# Autodesk Inventor assembly: Assembly
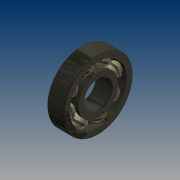
[picture p0: Inventor's stored thumbnail of the model, 180x180]
Saved by Autodesk Inventor 2014 (Build 180170000, 170)
## iProperties
Created: 2021-03-19
Part Number: Assembly
Document SubType Name: Assembly
Designer: Think Station
Author: Think Station
## Documents named in this file (5)
- E:\Entraco_Diptanshu\3D\##TEST##\Ball Bearing\Assembly.iam
- E:\Entraco_Diptanshu\3D\##TEST##\Ball Bearing\Outer Ring.ipt
- E:\Entraco_Diptanshu\3D\##TEST##\Ball Bearing\Inner Ring.ipt
- E:\Entraco_Diptanshu\3D\##TEST##\Ball Bearing\Ball.ipt
- E:\Entraco_Diptanshu\3D\##TEST##\Ball Bearing\Cage.ipt
## Components (12 placed, 4 different names)
1. Outer Ring:1 — Mate:1, Mate:2, Flush:1
2. Inner Ring:1 — Mate:3, Flush:1, Tangent:1, Mate:5, Angle:1
3. Cage:1 — Mate:7, Mate:8, Mate:9, Mate:11
4. Cage:2 — Flush:2, Mate:10, Mate:11
5. Ball:1 — Mate:4, Tangent:1, Mate:5, Mate:8
6. Ball:2
7. Ball:3
8. Ball:4
9. Ball:5
10. Ball:6
11. Ball:7
12. Ball:8
## Component patterns: (8 elements, first: Ball:1)
## Relationships (14: Mate 10, Flush 2, Tangent 1, Angle 1)
- Mate:1: Outer Ring:1
- Mate:2: Outer Ring:1
- Mate:3: Inner Ring:1
- Flush:1: Outer Ring:1 ↔ Inner Ring:1
- Mate:4: Ball:1
- Tangent:1: Inner Ring:1 ↔ Ball:1
- Mate:5: Inner Ring:1 ↔ Ball:1
- Mate:7: Cage:1
- Mate:8: Cage:1 ↔ Ball:1
- Mate:9: Cage:1
- Flush:2: Cage:2
- Mate:10: Cage:2
- Mate:11: Cage:1 ↔ Cage:2
- Angle:1 (60 deg): Inner Ring:1
